# Autodesk Inventor assembly: weldements2
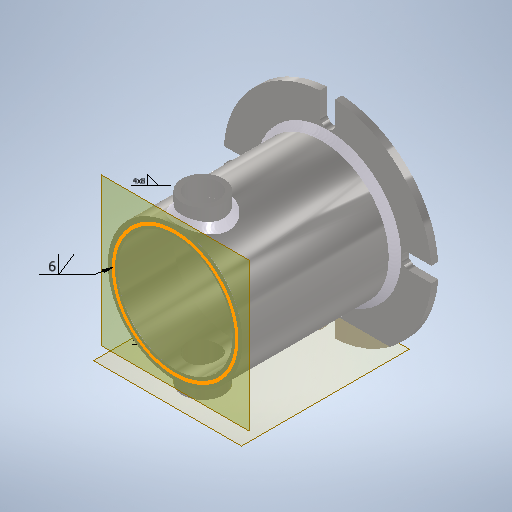
[picture p0: Inventor's stored thumbnail of the model, 512x512]
Saved by Autodesk Inventor 2025.2 (Build 292293000, 293)
## iProperties
Created: 2025-03-25
Part Number: weldements2
Document SubType Name: Weldment
Designer: bless
Weld Material: Welded Aluminum-6061
Author: bless
## Documents named in this file (6)
- C:\Users\bless\OneDrive - Conestoga College\Documents\Inventor\8071W25\weldmants\weldements2.iam
- C:\Users\bless\OneDrive - Conestoga College\Documents\Inventor\8071W25\weldmants\base.ipt
- C:\Users\bless\OneDrive - Conestoga College\Documents\Inventor\8071W25\weldmants\cylinder1.ipt
- C:\Users\bless\OneDrive - Conestoga College\Documents\Inventor\8071W25\weldmants\Part6.ipt
- C:\Users\bless\OneDrive - Conestoga College\Documents\Inventor\8071W25\weldmants\Part7.ipt
- C:\Users\bless\OneDrive - Conestoga College\Documents\Inventor\8071W25\weldmants\Part7_MIR.ipt
## Components (5 placed, 5 different names)
1. base:1 — Flush:1
2. cylinder1:1 — Flush:1, Flush:2, Flush:3, Flush:4, Flush:8
3. Part6:1 — Flush:2, Flush:3
4. Part7:1 — Flush:6, Flush:7, Flush:8
5. Part7_MIR:1 — Mate:1, Mate:2
## Relationships (10: Flush 8, Mate 2)
- Flush:1: base:1 ↔ cylinder1:1
- Flush:2: cylinder1:1 ↔ Part6:1
- Flush:3: cylinder1:1 ↔ Part6:1
- Flush:4 (-35.106 mm): cylinder1:1
- Flush:5 (120 mm)
- Flush:6: Part7:1
- Flush:7: Part7:1
- Flush:8: cylinder1:1 ↔ Part7:1
- Mate:1: Part7_MIR:1
- Mate:2: Part7_MIR:1
